# Autodesk Inventor assembly: Outer
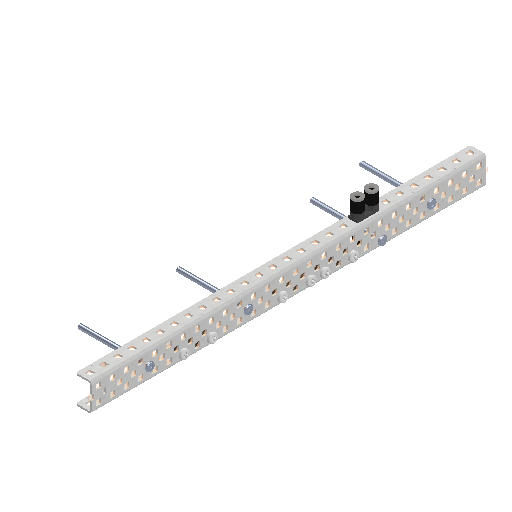
[picture p0: Inventor's stored thumbnail of the model, 512x512]
Saved by Autodesk Inventor 2025 (Build 290162000, 162)
## iProperties
Created: 2025-01-27
Part Number: Outer
Document SubType Name: Assembly
Designer: Averey Ku
Author: Averey Ku
## Documents named in this file (19)
- D:\VEX\High Stakes\CAD\V5\Chassis\Drivebay Right\Outer.iam
- D:\VEX\High Stakes\CAD\V5\Chassis\Drivebay Right\Bearing Flat Low Profile.ipt
- D:\VEX\High Stakes\CAD\V5\Chassis\Drivebay Right\NScrew Pan Head Threaded .500.ipt
- D:\VEX\High Stakes\CAD\ROBOPROS-CAD-Inventor\Structure\Hardware\Screw Steel - Star\SScrew Star Smooth 2.500.ipt
- D:\VEX\High Stakes\CAD\ROBOPROS-CAD-Inventor\Structure\Hardware\Screw Steel - Star.ipt
- D:\VEX\High Stakes\CAD\V5\Chassis\Drivebay Right\Nut Keps.ipt
- D:\VEX\High Stakes\CAD\ROBOPROS-CAD-Inventor\Structure\Hardware\Nut Nylon\Nut Nylon - White.ipt
- D:\VEX\High Stakes\CAD\ROBOPROS-CAD-Inventor\Structure\Hardware\Nut Nylon.ipt
- D:\VEX\High Stakes\CAD\V5\Chassis\Drivebay Right\Alu C 1x2x1x28.ipt
- D:\VEX\High Stakes\CAD\ROBOPROS-CAD-Inventor\Modified Parts\Bearing Flat Low Profile 2-Hole.ipt
- D:\VEX\High Stakes\CAD\ROBOPROS-CAD-Inventor\Motion\Spacers\Spacer Nylon .375 OD\NSpacer .375 OD x .375.ipt
- D:\VEX\High Stakes\CAD\ROBOPROS-CAD-Inventor\Motion\Spacers\Spacer Nylon .375 OD.ipt
- D:\VEX\High Stakes\CAD\ROBOPROS-CAD-Inventor\Motion\Spacers\Washer Steel\SWasher .375 OD x .062500.ipt
- D:\VEX\High Stakes\CAD\ROBOPROS-CAD-Inventor\Motion\Spacers\Washer Steel.ipt
- D:\VEX\High Stakes\CAD\ROBOPROS-CAD-Inventor\Structure\Standoff\Standoff .875.ipt
- D:\VEX\High Stakes\CAD\ROBOPROS-CAD-Inventor\Structure\Standoff.ipt
- D:\VEX\High Stakes\CAD\ROBOPROS-CAD-Inventor\Structure\Hardware\Screw Alu - Slotted\AScrew Slotted Threaded .250.ipt
- D:\VEX\High Stakes\CAD\ROBOPROS-CAD-Inventor\Structure\C Channel\Aluminum 1x2x1\Alu C 1x2x1x27.ipt
- D:\VEX\High Stakes\CAD\ROBOPROS-CAD-Inventor\Structure\Nylon Standoff Rounded\Nylon Standoff .875.ipt
## Components (32 placed, 13 different names)
1. Bearing Flat Low Profile:2 — Insert:21, Insert:22, Mate:3, Insert:32
2. Bearing Flat Low Profile:3 — Insert:23, Insert:24, Insert:44
3. NScrew Pan Head Threaded .500:2 — Insert:35
4. NScrew Pan Head Threaded .500:3 — Insert:37
5. NScrew Pan Head Threaded .500:4 — Insert:36
6. NScrew Pan Head Threaded .500:5 — Mate:4, Insert:39
7. NScrew Pan Head Threaded .500:6 — Insert:38
8. SScrew Star Smooth 2.500:1 — Insert:27
9. SScrew Star Smooth 2.500:2 — Insert:26
10. SScrew Star Smooth 2.500:3 — Insert:25
11. Nut Keps:1 — Insert:43
12. Nut Keps:2 — Insert:41
13. Nut Keps:3 — Insert:42
14. Nut Nylon - White:2 — Insert:21
15. Nut Nylon - White:4 — Insert:22
16. Nut Nylon - White:5 — Mate:4, Insert:23
17. Nut Nylon - White:6 — Insert:24
18. Alu C 1x2x1x28:1 — Insert:44, Insert:43, Insert:42, Insert:41, Insert:39, Insert:38, Insert:37, Insert:36, Insert:35, Mate:3, Insert:32, Insert:27, Insert:26, Insert:25, Flush:3, Flush:2, Flush:1, Mate:2, Insert:31, Insert:40, Insert:27, Insert:32, Mate:6, Insert:33, Insert:34, Insert:35, Mate:7
19. Bearing Flat Low Profile:4 — Mate:2, Insert:31, Insert:29, Insert:30
20. Nut Nylon - White:7 — Insert:29
21. Nut Nylon - White:8 — Insert:30
22. NScrew Pan Head Threaded .500:8 — Insert:40
23. SScrew Star Smooth 2.500:4 — Insert:27
24. Bearing Flat Low Profile 2-Hole:1 — Insert:32
25. NSpacer .375 OD x .375:1
26. SWasher .375 OD x .062500:1
27. NSpacer .375 OD x .375:2 — Mate:6
28. SWasher .375 OD x .062500:2
29. Standoff .875:1 — Insert:33
30. AScrew Slotted Threaded .250:1 — Insert:34
31. Alu C 1x2x1x27:1 — Insert:35, Mate:7, Insert:36
32. Nylon Standoff .875:1 — Insert:36
## Relationships (39: Insert 31, Mate 6, Flush 2)
- Insert:21 (1.27 mm): Bearing Flat Low Profile:2 ↔ Nut Nylon - White:2
- Insert:22 (1.27 mm): Bearing Flat Low Profile:2 ↔ Nut Nylon - White:4
- Mate:4: NScrew Pan Head Threaded .500:5 ↔ Nut Nylon - White:5
- Insert:23 (1.27 mm): Bearing Flat Low Profile:3 ↔ Nut Nylon - White:5
- Insert:24 (1.27 mm): Bearing Flat Low Profile:3 ↔ Nut Nylon - White:6
- Insert:44: Bearing Flat Low Profile:3 ↔ Alu C 1x2x1x28:1
- Insert:43: Nut Keps:1 ↔ Alu C 1x2x1x28:1
- Insert:42: Nut Keps:3 ↔ Alu C 1x2x1x28:1
- Insert:41: Nut Keps:2 ↔ Alu C 1x2x1x28:1
- Insert:39: NScrew Pan Head Threaded .500:5 ↔ Alu C 1x2x1x28:1
- Insert:38: NScrew Pan Head Threaded .500:6 ↔ Alu C 1x2x1x28:1
- Insert:37: NScrew Pan Head Threaded .500:3 ↔ Alu C 1x2x1x28:1
- Insert:36: NScrew Pan Head Threaded .500:4 ↔ Alu C 1x2x1x28:1
- Insert:35: NScrew Pan Head Threaded .500:2 ↔ Alu C 1x2x1x28:1
- Mate:3: Bearing Flat Low Profile:2 ↔ Alu C 1x2x1x28:1
- Insert:32: Bearing Flat Low Profile:2 ↔ Alu C 1x2x1x28:1
- Insert:27 (1.5875 mm): SScrew Star Smooth 2.500:1 ↔ Alu C 1x2x1x28:1
- Insert:26 (1.5875 mm): SScrew Star Smooth 2.500:2 ↔ Alu C 1x2x1x28:1
- Insert:25 (1.5875 mm): SScrew Star Smooth 2.500:3 ↔ Alu C 1x2x1x28:1
- Flush:3: Alu C 1x2x1x28:1
- Flush:2 (-12.7 mm): Alu C 1x2x1x28:1
- Flush:1 [Mate] (-177.8 mm): Alu C 1x2x1x28:1
- Mate:2: Alu C 1x2x1x28:1 ↔ Bearing Flat Low Profile:4
- Insert:31: Alu C 1x2x1x28:1 ↔ Bearing Flat Low Profile:4
- Insert:29 (1.27 mm): Bearing Flat Low Profile:4 ↔ Nut Nylon - White:7
- Insert:30 (1.27 mm): Bearing Flat Low Profile:4 ↔ Nut Nylon - White:8
- Insert:40: Alu C 1x2x1x28:1 ↔ NScrew Pan Head Threaded .500:8
- Insert:27 (1.5875 mm): Alu C 1x2x1x28:1 ↔ SScrew Star Smooth 2.500:4
- [Insert]: NSpacer .375 OD x .375:1 ↔ SWasher .375 OD x .062500:1
- [Insert] (1.27 mm): Bearing Flat Low Profile 2-Hole:1 ↔ NSpacer .375 OD x .375:1
- [Insert]: NSpacer .375 OD x .375:2 ↔ SWasher .375 OD x .062500:2
- [Insert] (1.27 mm): Bearing Flat Low Profile 2-Hole:1 ↔ NSpacer .375 OD x .375:2
- Insert:32: Alu C 1x2x1x28:1 ↔ Bearing Flat Low Profile 2-Hole:1
- Mate:6: Alu C 1x2x1x28:1 ↔ NSpacer .375 OD x .375:2
- Insert:33: Alu C 1x2x1x28:1 ↔ Standoff .875:1
- Insert:34: Alu C 1x2x1x28:1 ↔ AScrew Slotted Threaded .250:1
- Insert:35: Alu C 1x2x1x28:1 ↔ Alu C 1x2x1x27:1
- Mate:7: Alu C 1x2x1x28:1 ↔ Alu C 1x2x1x27:1
- Insert:36: Alu C 1x2x1x27:1 ↔ Nylon Standoff .875:1
## Named parameters: d102_d100 = 0 mm
